# Autodesk Inventor assembly: ElvFrontFrame
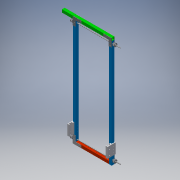
[picture p0: Inventor's stored thumbnail of the model, 180x180]
Saved by Autodesk Inventor 2019 (Build 230136000, 136)
## iProperties
Created: 2019-01-10
Part Number: ElvFrontFrame
Document SubType Name: Assembly
Designer: james
Mass: 1675.61 g
Surface Area: 6085.53 cm^2
Volume: 594.432 cm^3
Density: 2.81883 g/cm^3
Author: james
## Documents named in this file (7)
- F:\JimsDesign\2019CHS4089\ElvFrontFrame.iam
- F:\JimsDesign\2019CHS4089\ElvCrossBeam.ipt
- F:\JimsDesign\2019CHS4089\ElvFrontBeam.ipt
- F:\JimsDesign\2019CHS4089\ElvShaft.iam
- F:\JimsDesign\2019CHS4089\ElvTopBeam.ipt
- F:\JimsDesign\2019CHS4089\elvRivetPlate.ipt
- F:\JimsDesign\2019CHS4089\ElvDelV6.ipt
## Components (15 placed, 6 different names)
1. ElvCrossBeam:1 — Mate:43, Mate:44, Mate:45, Mate:46, Mate:47, Mate:48
2. ElvFrontBeam:1 — Mate:22, Flush:17, Flush:21, Mate:30, Flush:24, Mate:37, Mate:38, Mate:39, Mate:62, Mate:63, Mate:64
3. ElvFrontBeam:2 — Mate:20, Mate:31, Mate:32, Mate:40, Mate:41, Mate:42, Mate:49, Mate:50, Mate:51, Mate:55, Mate:56, Mate:57, Mate:59, Mate:60, Mate:61
4. ElvDelV6:1 — Mate:62, Mate:63, Mate:64
5. ElvDelV6:2 — Mate:59, Mate:60, Mate:61
6. ElvShaft:1 [sub-assembly] — Mate:22, Mate:32
7. ElvShaft:2 [sub-assembly] — Mate:20, Mate:31
8. ElvTopBeam:1 — Mate:52, Mate:53, Mate:54
9. elvRivetPlate:1 — Mate:55, Mate:56, Mate:57
10. elvRivetPlate:2 — Flush:21
11. elvRivetPlate:3 — Flush:17
12. elvRivetPlate:4 — Mate:49, Mate:50, Mate:51, Mate:52, Mate:53, Mate:54
13. elvRivetPlate:5 — Mate:30, Flush:24, Mate:43
14. elvRivetPlate:6 — Mate:37, Mate:38, Mate:39, Mate:44, Mate:45
15. elvRivetPlate:7 — Mate:40, Mate:41, Mate:42, Mate:46, Mate:47, Mate:48
## Relationships (35: Mate 32, Flush 3)
- Mate:20: ElvFrontBeam:2 ↔ ElvShaft:2
- Mate:22: ElvFrontBeam:1 ↔ ElvShaft:1
- Flush:17: ElvFrontBeam:1 ↔ elvRivetPlate:3
- Flush:21: ElvFrontBeam:1 ↔ elvRivetPlate:2
- Mate:30: ElvFrontBeam:1 ↔ elvRivetPlate:5
- Flush:24: ElvFrontBeam:1 ↔ elvRivetPlate:5
- Mate:31: ElvFrontBeam:2 ↔ ElvShaft:2
- Mate:32: ElvFrontBeam:2 ↔ ElvShaft:1
- Mate:37: ElvFrontBeam:1 ↔ elvRivetPlate:6
- Mate:38: ElvFrontBeam:1 ↔ elvRivetPlate:6
- Mate:39: ElvFrontBeam:1 ↔ elvRivetPlate:6
- Mate:40: ElvFrontBeam:2 ↔ elvRivetPlate:7
- Mate:41: ElvFrontBeam:2 ↔ elvRivetPlate:7
- Mate:42: ElvFrontBeam:2 ↔ elvRivetPlate:7
- Mate:43: ElvCrossBeam:1 ↔ elvRivetPlate:5
- Mate:44: ElvCrossBeam:1 ↔ elvRivetPlate:6
- Mate:45: ElvCrossBeam:1 ↔ elvRivetPlate:6
- Mate:46: ElvCrossBeam:1 ↔ elvRivetPlate:7
- Mate:47: ElvCrossBeam:1 ↔ elvRivetPlate:7
- Mate:48: ElvCrossBeam:1 ↔ elvRivetPlate:7
- Mate:49: ElvFrontBeam:2 ↔ elvRivetPlate:4
- Mate:50: ElvFrontBeam:2 ↔ elvRivetPlate:4
- Mate:51: ElvFrontBeam:2 ↔ elvRivetPlate:4
- Mate:52: ElvTopBeam:1 ↔ elvRivetPlate:4
- Mate:53: ElvTopBeam:1 ↔ elvRivetPlate:4
- Mate:54: ElvTopBeam:1 ↔ elvRivetPlate:4
- Mate:55: ElvFrontBeam:2 ↔ elvRivetPlate:1
- Mate:56: ElvFrontBeam:2 ↔ elvRivetPlate:1
- Mate:57: ElvFrontBeam:2 ↔ elvRivetPlate:1
- Mate:59: ElvFrontBeam:2 ↔ ElvDelV6:2
- Mate:60: ElvFrontBeam:2 ↔ ElvDelV6:2
- Mate:61: ElvFrontBeam:2 ↔ ElvDelV6:2
- Mate:62: ElvFrontBeam:1 ↔ ElvDelV6:1
- Mate:63: ElvFrontBeam:1 ↔ ElvDelV6:1
- Mate:64: ElvFrontBeam:1 ↔ ElvDelV6:1
